# Autodesk Inventor assembly: steering assembly v1
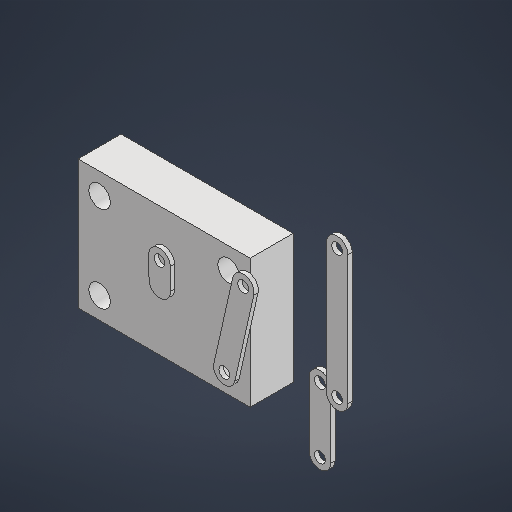
[picture p0: Inventor's stored thumbnail of the model, 512x512]
Saved by Autodesk Inventor 2026.1 (Build 301233000, 233)
## iProperties
Created: 2026-06-10
Part Number: steering assembly v1
Document SubType Name: Assembly
Designer: share
Author: share
## Documents named in this file (6)
- C:\Users\share\OneDrive\Documents\Personal Projects\GOGO Kart\CAD\GOGO_KART_FSAE\Shareef\Suspension Parts\Steering\steering assembly v1.iam
- C:\Users\share\OneDrive\Documents\Personal Projects\GOGO Kart\CAD\GOGO_KART_FSAE\Shareef\Suspension Parts\Steering\center block.ipt
- C:\Users\share\OneDrive\Documents\Personal Projects\GOGO Kart\CAD\GOGO_KART_FSAE\Shareef\Suspension Parts\Steering\main rack connection.ipt
- C:\Users\share\OneDrive\Documents\Personal Projects\GOGO Kart\CAD\GOGO_KART_FSAE\Shareef\Suspension Parts\Steering\arm.ipt
- C:\Users\share\OneDrive\Documents\Personal Projects\GOGO Kart\CAD\GOGO_KART_FSAE\Shareef\Suspension Parts\Steering\arm 1.ipt
- C:\Users\share\OneDrive\Documents\Personal Projects\GOGO Kart\CAD\GOGO_KART_FSAE\Shareef\Suspension Parts\Steering\arm 2.ipt
## Components (5 placed, 5 different names)
1. center block:1 — Insert:1, Flush:1, Flush:2, Flush:3, Insert:2
2. main rack connection:1 — Insert:1
3. arm:1 — Insert:2
4. arm 1:1
5. arm 2:1
## Relationships (5: Flush 3, Insert 2)
- Insert:1: center block:1 ↔ main rack connection:1
- Flush:1: center block:1
- Flush:2: center block:1
- Flush:3: center block:1
- Insert:2: center block:1 ↔ arm:1
